# Autodesk Inventor assembly: SuctionblockDelcotec
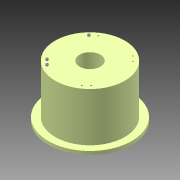
[picture p0: Inventor's stored thumbnail of the model, 180x180]
Saved by Autodesk Inventor 2013 (Build 170138000, 138)
## iProperties
Created: 2014-01-06
Part Number: SuctionblockDelcotec
Document SubType Name: Assembly
Designer: Frank Meier
Author: Frank Meier
## Documents named in this file (3)
- C:\Users\Frank Meier\Documents\Inventor\Delvotec-Saugplatte\SuctionblockDelcotec.iam
- C:\Users\Frank Meier\Documents\Inventor\Delvotec-Saugplatte\Delvotec-Saughalterung.ipt
- C:\Users\Frank Meier\Documents\Inventor\Content Center Files\R2013\de-DE\ISO 4762(2)\ISO 4762 - M4 x 8ISO.ipt
## Components (4 placed, 2 different names)
1. Delvotec-Saughalterung:1 — Einfügen:1, Einfügen:2, Einfügen:3
2. ISO 4762 M4 x 8:1 — Einfügen:3
3. ISO 4762 M4 x 8:2 — Einfügen:1
4. ISO 4762 M4 x 8:3 — Einfügen:2
## Relationships (3: Insert 3)
- Einfügen:1 [Insert]: Delvotec-Saughalterung:1 ↔ ISO 4762 M4 x 8:2
- Einfügen:2 [Insert]: Delvotec-Saughalterung:1 ↔ ISO 4762 M4 x 8:3
- Einfügen:3 [Insert]: Delvotec-Saughalterung:1 ↔ ISO 4762 M4 x 8:1
